# Autodesk Inventor assembly: X-Gantry Joinder Right Assembly
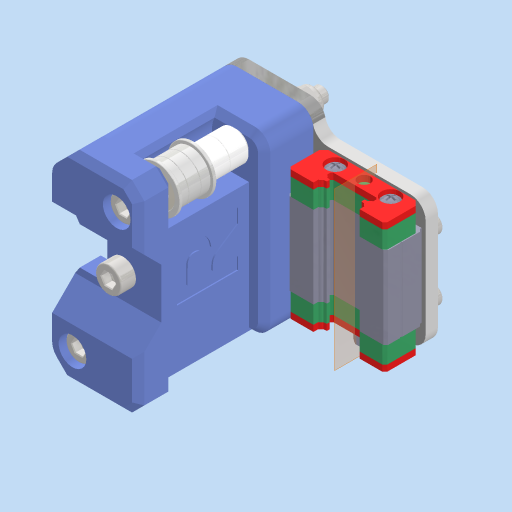
[picture p0: Inventor's stored thumbnail of the model, 512x512]
Saved by Autodesk Inventor 2023.2 (Build 272271000, 271)
## iProperties
Created: 2023-11-28
Part Number: X-Gantry Joinder Right Assembly
Document SubType Name: Assembly
Designer: Nils Bade
Author: Nils Bade
## Documents named in this file (14)
- C:\Users\nilsb\Documents\Inventor\Projektarbeit-Bade\RatRig_Bade\X-Gantry Joinder Right Assembly.iam
- C:\Users\nilsb\Documents\Inventor\Projektarbeit-Bade\RatRig_modified\XY Joiner Plate for 4040.ipt
- C:\Users\nilsb\Documents\Inventor\Projektarbeit-Bade\RatRig_modified\MGN15 Linear-Rail-Block.ipt
- C:\Users\nilsb\Documents\Inventor\Projektarbeit-Bade\Schrauben\Cap Head Screw M5x12 v2.ipt
- C:\Users\nilsb\Documents\Inventor\Projektarbeit-Bade\Schrauben\Cap Head Screw M3x12 v2.ipt
- C:\Users\nilsb\Documents\Inventor\Projektarbeit-Bade\Schrauben\Cap Head Screw M5x10 v2.ipt
- C:\Users\nilsb\Documents\Inventor\Projektarbeit-Bade\RatRig_Standards\T-Nut - Square type for 2020 - M5 v2.ipt
- C:\Users\nilsb\Documents\Inventor\Projektarbeit-Bade\Schrauben\Cap Head Screw M5x60.ipt
- C:\Users\nilsb\Documents\Inventor\Projektarbeit-Bade\RatRig_Standards\Hex Locking Nut - M5 v2.ipt
- C:\Users\nilsb\Documents\Inventor\Projektarbeit-Bade\RatRig_Standards\Mini Precision Shim - 8x5x1mm v2.ipt
- C:\Users\nilsb\Documents\Inventor\Projektarbeit-Bade\RatRig_Standards\Ball Bearing - 695ZZ v1.ipt
- C:\Users\nilsb\Documents\Inventor\Projektarbeit-Bade\RatRig_Standards\Ball Bearing - F695ZZ v1.ipt
- C:\Users\nilsb\Documents\Inventor\Projektarbeit-Bade\RatRig_Standards\Aluminium Spacer - 6mm v2.ipt
- C:\Users\nilsb\Documents\Inventor\Projektarbeit-Bade\RatRig_modified\xy Joiner Right for 4040 V1.ipt
## Components (33 placed, 13 different names)
1. xy Joiner Right for 4040:2
2. XY Joiner Plate for 4040:1 — Passend:4, Passend:5, Passend:6, Passend:7, Passend:8, Passend:9, Passend:10, Passend:11, Passend:12, Passend:13, Passend:14, Passend:33, Passend:34
3. MGN15 Linear-Rail-Block:1 — Passend:4, Passend:5, Passend:6
4. Cap Head Screw M3x12 v2:1 — Passend:7, Passend:11
5. Cap Head Screw M3x12 v2:2 — Passend:8, Passend:12
6. Cap Head Screw M3x12 v2:3 — Passend:9, Passend:13
7. Cap Head Screw M3x12 v2:4 — Passend:10, Passend:14
8. Cap Head Screw M5x10 v2:1
9. Cap Head Screw M5x10 v2:2
10. Cap Head Screw M5x12 v2:1
11. T-Nut - Square type for 2020 - M5 v2:1
12. T-Nut - Square type for 2020 - M5 v2:2
13. T-Nut - Square type for 2020 - M5 v2:3
14. Cap Head Screw M5x60:1 — Passend:31, Passend:51, Passend:53, Passend:55, Passend:57, Passend:59, Passend:61, Passend:63, Passend:65
15. Cap Head Screw M5x60:2 — Passend:32, Passend:35, Passend:37, Passend:39, Passend:41, Passend:43, Passend:45, Passend:47, Passend:49
16. Hex Locking Nut - M5 v2:1 — Passend:31, Passend:34
17. Hex Locking Nut - M5 v2:2 — Passend:32, Passend:33
18. Mini Precision Shim - 8x5x1mm v2:1 — Passend:35, Passend:38
19. Mini Precision Shim - 8x5x1mm v2:2 — Passend:49, Passend:50
20. Mini Precision Shim - 8x5x1mm v2:3 — Passend:41, Passend:42, Passend:44
21. Mini Precision Shim - 8x5x1mm v2:4 — Passend:65, Passend:66
22. Mini Precision Shim - 8x5x1mm v2:5 — Passend:59, Passend:60, Passend:62
23. Mini Precision Shim - 8x5x1mm v2:6 — Passend:51, Passend:54
24. Ball Bearing - 695ZZ v1:1 — Passend:45, Passend:46, Passend:48
25. Ball Bearing - 695ZZ v1:2 — Passend:55, Passend:56, Passend:58
26. Ball Bearing - F695ZZ v1:1 — Passend:43, Passend:44, Passend:46
27. Ball Bearing - F695ZZ v1:2 — Passend:53, Passend:54, Passend:56
28. Ball Bearing - F695ZZ v1:3 — Passend:47, Passend:48, Passend:50
29. Ball Bearing - F695ZZ v1:4 — Passend:57, Passend:58, Passend:60
30. Aluminium Spacer - 6mm v2:1 — Passend:37, Passend:38, Passend:40
31. Aluminium Spacer - 6mm v2:2 — Passend:39, Passend:40, Passend:42
32. Aluminium Spacer - 6mm v2:3 — Passend:63, Passend:64, Passend:66
33. Aluminium Spacer - 6mm v2:4 — Passend:61, Passend:62, Passend:64
## Relationships (69: Mate 66, Angle 3)
- [Mate]: xy Joiner Right for 4040:2 ↔ XY Joiner Plate for 4040:1
- [Mate]: xy Joiner Right for 4040:2 ↔ XY Joiner Plate for 4040:1
- [Mate]: xy Joiner Right for 4040:2 ↔ XY Joiner Plate for 4040:1
- Passend:4 [Mate]: XY Joiner Plate for 4040:1 ↔ MGN15 Linear-Rail-Block:1
- Passend:5 [Mate]: XY Joiner Plate for 4040:1 ↔ MGN15 Linear-Rail-Block:1
- Passend:6 [Mate]: XY Joiner Plate for 4040:1 ↔ MGN15 Linear-Rail-Block:1
- Passend:7 [Mate]: XY Joiner Plate for 4040:1 ↔ Cap Head Screw M3x12 v2:1
- Passend:8 [Mate]: XY Joiner Plate for 4040:1 ↔ Cap Head Screw M3x12 v2:2
- Passend:9 [Mate]: XY Joiner Plate for 4040:1 ↔ Cap Head Screw M3x12 v2:3
- Passend:10 [Mate]: XY Joiner Plate for 4040:1 ↔ Cap Head Screw M3x12 v2:4
- Passend:11 [Mate]: XY Joiner Plate for 4040:1 ↔ Cap Head Screw M3x12 v2:1
- Passend:12 [Mate]: XY Joiner Plate for 4040:1 ↔ Cap Head Screw M3x12 v2:2
- Passend:13 [Mate]: XY Joiner Plate for 4040:1 ↔ Cap Head Screw M3x12 v2:3
- Passend:14 [Mate]: XY Joiner Plate for 4040:1 ↔ Cap Head Screw M3x12 v2:4
- [Mate]: xy Joiner Right for 4040:2 ↔ T-Nut - Square type for 2020 - M5 v2:2
- [Mate]: xy Joiner Right for 4040:2 ↔ T-Nut - Square type for 2020 - M5 v2:3
- [Mate]: xy Joiner Right for 4040:2 ↔ T-Nut - Square type for 2020 - M5 v2:1
- [Angle] (0 deg): xy Joiner Right for 4040:2 ↔ T-Nut - Square type for 2020 - M5 v2:1
- [Angle] (0 deg): xy Joiner Right for 4040:2 ↔ T-Nut - Square type for 2020 - M5 v2:2
- [Angle] (0 deg): xy Joiner Right for 4040:2 ↔ T-Nut - Square type for 2020 - M5 v2:3
- [Mate] (1.8 mm): xy Joiner Right for 4040:2 ↔ T-Nut - Square type for 2020 - M5 v2:3
- [Mate] (1.8 mm): xy Joiner Right for 4040:2 ↔ T-Nut - Square type for 2020 - M5 v2:2
- [Mate] (1.8 mm): xy Joiner Right for 4040:2 ↔ T-Nut - Square type for 2020 - M5 v2:1
- [Mate]: xy Joiner Right for 4040:2 ↔ Cap Head Screw M5x10 v2:1
- [Mate]: xy Joiner Right for 4040:2 ↔ Cap Head Screw M5x10 v2:1
- [Mate]: xy Joiner Right for 4040:2 ↔ Cap Head Screw M5x10 v2:2
- [Mate]: xy Joiner Right for 4040:2 ↔ Cap Head Screw M5x10 v2:2
- [Mate]: xy Joiner Right for 4040:2 ↔ Cap Head Screw M5x12 v2:1
- [Mate]: xy Joiner Right for 4040:2 ↔ Cap Head Screw M5x12 v2:1
- [Mate]: xy Joiner Right for 4040:2 ↔ Cap Head Screw M5x60:1
- [Mate]: xy Joiner Right for 4040:2 ↔ Cap Head Screw M5x60:2
- [Mate]: xy Joiner Right for 4040:2 ↔ Cap Head Screw M5x60:2
- [Mate]: xy Joiner Right for 4040:2 ↔ Cap Head Screw M5x60:1
- Passend:31 [Mate]: Cap Head Screw M5x60:1 ↔ Hex Locking Nut - M5 v2:1
- Passend:32 [Mate]: Cap Head Screw M5x60:2 ↔ Hex Locking Nut - M5 v2:2
- Passend:33 [Mate]: XY Joiner Plate for 4040:1 ↔ Hex Locking Nut - M5 v2:2
- Passend:34 [Mate]: XY Joiner Plate for 4040:1 ↔ Hex Locking Nut - M5 v2:1
- Passend:35 [Mate]: Cap Head Screw M5x60:2 ↔ Mini Precision Shim - 8x5x1mm v2:1
- [Mate]: xy Joiner Right for 4040:2 ↔ Mini Precision Shim - 8x5x1mm v2:1
- Passend:37 [Mate]: Cap Head Screw M5x60:2 ↔ Aluminium Spacer - 6mm v2:1
- Passend:38 [Mate]: Mini Precision Shim - 8x5x1mm v2:1 ↔ Aluminium Spacer - 6mm v2:1
- Passend:39 [Mate]: Cap Head Screw M5x60:2 ↔ Aluminium Spacer - 6mm v2:2
- Passend:40 [Mate]: Aluminium Spacer - 6mm v2:1 ↔ Aluminium Spacer - 6mm v2:2
- Passend:41 [Mate]: Cap Head Screw M5x60:2 ↔ Mini Precision Shim - 8x5x1mm v2:3
- Passend:42 [Mate]: Mini Precision Shim - 8x5x1mm v2:3 ↔ Aluminium Spacer - 6mm v2:2
- Passend:43 [Mate]: Cap Head Screw M5x60:2 ↔ Ball Bearing - F695ZZ v1:1
- Passend:44 [Mate]: Mini Precision Shim - 8x5x1mm v2:3 ↔ Ball Bearing - F695ZZ v1:1
- Passend:45 [Mate]: Cap Head Screw M5x60:2 ↔ Ball Bearing - 695ZZ v1:1
- Passend:46 [Mate]: Ball Bearing - 695ZZ v1:1 ↔ Ball Bearing - F695ZZ v1:1
- Passend:47 [Mate]: Cap Head Screw M5x60:2 ↔ Ball Bearing - F695ZZ v1:3
- Passend:48 [Mate]: Ball Bearing - 695ZZ v1:1 ↔ Ball Bearing - F695ZZ v1:3
- Passend:49 [Mate]: Cap Head Screw M5x60:2 ↔ Mini Precision Shim - 8x5x1mm v2:2
- Passend:50 [Mate]: Mini Precision Shim - 8x5x1mm v2:2 ↔ Ball Bearing - F695ZZ v1:3
- Passend:51 [Mate]: Cap Head Screw M5x60:1 ↔ Mini Precision Shim - 8x5x1mm v2:6
- [Mate]: xy Joiner Right for 4040:2 ↔ Mini Precision Shim - 8x5x1mm v2:6
- Passend:53 [Mate]: Cap Head Screw M5x60:1 ↔ Ball Bearing - F695ZZ v1:2
- Passend:54 [Mate]: Mini Precision Shim - 8x5x1mm v2:6 ↔ Ball Bearing - F695ZZ v1:2
- Passend:55 [Mate]: Cap Head Screw M5x60:1 ↔ Ball Bearing - 695ZZ v1:2
- Passend:56 [Mate]: Ball Bearing - 695ZZ v1:2 ↔ Ball Bearing - F695ZZ v1:2
- Passend:57 [Mate]: Cap Head Screw M5x60:1 ↔ Ball Bearing - F695ZZ v1:4
- Passend:58 [Mate]: Ball Bearing - 695ZZ v1:2 ↔ Ball Bearing - F695ZZ v1:4
- Passend:59 [Mate]: Cap Head Screw M5x60:1 ↔ Mini Precision Shim - 8x5x1mm v2:5
- Passend:60 [Mate]: Mini Precision Shim - 8x5x1mm v2:5 ↔ Ball Bearing - F695ZZ v1:4
- Passend:61 [Mate]: Cap Head Screw M5x60:1 ↔ Aluminium Spacer - 6mm v2:4
- Passend:62 [Mate]: Mini Precision Shim - 8x5x1mm v2:5 ↔ Aluminium Spacer - 6mm v2:4
- Passend:63 [Mate]: Cap Head Screw M5x60:1 ↔ Aluminium Spacer - 6mm v2:3
- Passend:64 [Mate]: Aluminium Spacer - 6mm v2:3 ↔ Aluminium Spacer - 6mm v2:4
- Passend:65 [Mate]: Cap Head Screw M5x60:1 ↔ Mini Precision Shim - 8x5x1mm v2:4
- Passend:66 [Mate]: Mini Precision Shim - 8x5x1mm v2:4 ↔ Aluminium Spacer - 6mm v2:3
